# Autodesk Inventor assembly: Assembly_Aisola
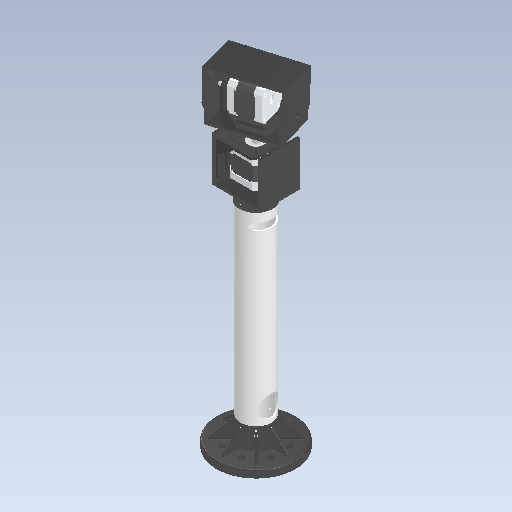
[picture p0: Inventor's stored thumbnail of the model, 512x512]
Saved by Autodesk Inventor 2025.1 (Build 291241000, 241)
## iProperties
Created: 2024-11-07
Part Number: Assembly_Aisola
Document SubType Name: Assembly
Designer: ramad
Author: ramad
## Documents named in this file (9)
- D:\MSIB\Aisola\Assembly_Aisola.iam
- D:\MSIB\Aisola\nema-17-45.snapshot.6\bawahbase.ipt
- D:\MSIB\Aisola\nema-17-45.snapshot.6\pvc30cm.ipt
- D:\MSIB\Aisola\nema-17-45.snapshot.6\Nema 17.ipt
- D:\MSIB\Aisola\baseatas.ipt
- D:\MSIB\Aisola\nema-17-23-stepper-motor-mounts-1.snapshot.6\NEMA 17 A-Body\NEMA 17 A-Body\NEMA 17 A-Body.ipt
- D:\MSIB\Aisola\mountingnema.ipt
- D:\MSIB\Aisola\baseatas2.ipt
- D:\MSIB\Aisola\atassolar.ipt
## Components (10 placed, 8 different names)
1. bawahbase:1 — Mate:1, Mate:2, Mate:3, Mate:4, Mate:5, Mate:6
2. pvc30cm:1 — Mate:4, Mate:5, Mate:6, Mate:10, Mate:11, Mate:12
3. Nema 17:1 — Mate:13, Mate:14, Flush:1, Mate:26, Mate:27
4. baseatas:1 — Mate:10, Mate:11, Mate:12, Mate:15, Mate:16, Flush:2
5. NEMA 17 A-Body:1 — Mate:13, Mate:14, Flush:1, Mate:15, Mate:16, Flush:2
6. mountingnema:1 — Mate:21, Flush:4, Mate:23, Mate:26, Flush:6
7. NEMA 17 A-Body:2 — Mate:19, Mate:20, Flush:3, Mate:24, Mate:25, Flush:5
8. Nema 17:2 — Mate:19, Mate:20, Flush:3
9. baseatas2:1 — Mate:21, Mate:22, Mate:23, Mate:24, Mate:25, Flush:5, Mate:28, Mate:29, Mate:30
10. atassolar:1 — Mate:28, Mate:29, Mate:30
## Relationships (31: Mate 25, Flush 6)
- Mate:1: bawahbase:1
- Mate:2: bawahbase:1
- Mate:3: bawahbase:1
- Mate:4: bawahbase:1 ↔ pvc30cm:1
- Mate:5: bawahbase:1 ↔ pvc30cm:1
- Mate:6: bawahbase:1 ↔ pvc30cm:1
- Mate:10: pvc30cm:1 ↔ baseatas:1
- Mate:11: pvc30cm:1 ↔ baseatas:1
- Mate:12: pvc30cm:1 ↔ baseatas:1
- Mate:13: Nema 17:1 ↔ NEMA 17 A-Body:1
- Mate:14: Nema 17:1 ↔ NEMA 17 A-Body:1
- Flush:1: Nema 17:1 ↔ NEMA 17 A-Body:1
- Mate:15: baseatas:1 ↔ NEMA 17 A-Body:1
- Mate:16: baseatas:1 ↔ NEMA 17 A-Body:1
- Flush:2: baseatas:1 ↔ NEMA 17 A-Body:1
- Mate:19: NEMA 17 A-Body:2 ↔ Nema 17:2
- Mate:20: NEMA 17 A-Body:2 ↔ Nema 17:2
- Flush:3: NEMA 17 A-Body:2 ↔ Nema 17:2
- Mate:21: mountingnema:1 ↔ baseatas2:1
- Flush:4: mountingnema:1
- Mate:22: baseatas2:1
- Mate:23: mountingnema:1 ↔ baseatas2:1
- Mate:24: NEMA 17 A-Body:2 ↔ baseatas2:1
- Mate:25: NEMA 17 A-Body:2 ↔ baseatas2:1
- Flush:5: NEMA 17 A-Body:2 ↔ baseatas2:1
- Mate:26: Nema 17:1 ↔ mountingnema:1
- Flush:6: mountingnema:1
- Mate:27: Nema 17:1
- Mate:28: baseatas2:1 ↔ atassolar:1
- Mate:29: baseatas2:1 ↔ atassolar:1
- Mate:30: baseatas2:1 ↔ atassolar:1
